# Autodesk Inventor assembly: Сборка сортировщика
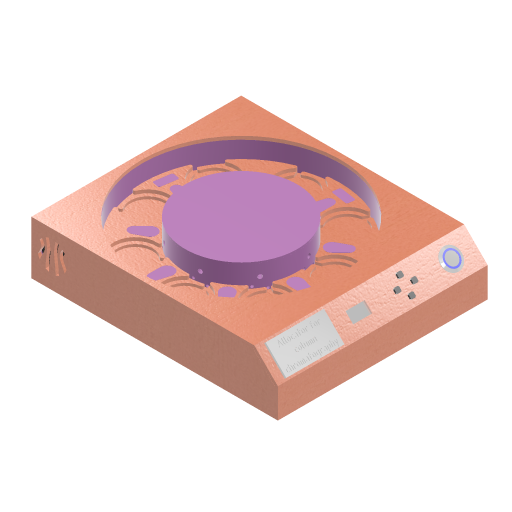
[picture p0: Inventor's stored thumbnail of the model, 512x512]
Saved by Autodesk Inventor 2024.1 (Build 281209000, 209)
## iProperties
Created: 2023-06-10
Part Number: Сборка сортировщика
Document SubType Name: Assembly
Designer: Admin
Mass: 1926.82 g
Surface Area: 9393.72 cm^2
Volume: 1926.82 cm^3
Density: 1 g/cm^3
Author: Admin
## Documents named in this file (27)
- C:\Users\aleks\OneDrive\Рабочий стол\Хроматографический сортировщик\Детали\Сборка сортировщика.iam
- C:\Users\aleks\OneDrive\Рабочий стол\Хроматографический сортировщик\Детали\Барабан в сборке.iam
- C:\Users\aleks\OneDrive\Рабочий стол\Хроматографический сортировщик\Детали\Корпус.ipt
- C:\Users\aleks\OneDrive\Рабочий стол\Хроматографический сортировщик\Детали\Покупные\Болт М3 12 мм.ipt
- C:\Users\aleks\OneDrive\Рабочий стол\Хроматографический сортировщик\Детали\Держатель динамика.ipt
- C:\Users\aleks\OneDrive\Рабочий стол\Хроматографический сортировщик\Детали\Лазерная установка.ipt
- C:\Users\aleks\OneDrive\Рабочий стол\Хроматографический сортировщик\Детали\Установка датчика холла.ipt
- C:\Users\aleks\OneDrive\Рабочий стол\Хроматографический сортировщик\Детали\Концентратор.ipt
- C:\Users\aleks\OneDrive\Рабочий стол\Хроматографический сортировщик\Детали\Покупные\Мотор.ipt
- C:\Users\aleks\OneDrive\Рабочий стол\Хроматографический сортировщик\Детали\Покупные\Плата главная.ipt
- C:\Users\aleks\OneDrive\Рабочий стол\Хроматографический сортировщик\Детали\Покупные\Болт М3 35мм.ipt
- C:\Users\aleks\OneDrive\Рабочий стол\Хроматографический сортировщик\Детали\Покупные\Болт М3 16 мм.ipt
- C:\Users\aleks\OneDrive\Рабочий стол\Хроматографический сортировщик\Детали\Покупные\Подшипник.ipt
- C:\Users\aleks\OneDrive\Рабочий стол\Хроматографический сортировщик\Детали\Покупные\Лазер.ipt
- C:\Users\aleks\OneDrive\Рабочий стол\Хроматографический сортировщик\Детали\Покупные\Лазер маленький.ipt
- C:\Users\aleks\OneDrive\Рабочий стол\Хроматографический сортировщик\Детали\Планетарная шестерня.ipt
- C:\Users\aleks\OneDrive\Рабочий стол\Хроматографический сортировщик\Детали\Шестерня малая.ipt
- C:\Users\aleks\OneDrive\Рабочий стол\Хроматографический сортировщик\Детали\Покупные\Вал.ipt
- C:\Users\aleks\OneDrive\Рабочий стол\Хроматографический сортировщик\Детали\Покупные\Болт М3 6 мм.ipt
- C:\Users\aleks\OneDrive\Рабочий стол\Хроматографический сортировщик\Детали\Покупные\Динамик.ipt
- C:\Users\aleks\OneDrive\Рабочий стол\Хроматографический сортировщик\Детали\Табличка.ipt
- C:\Users\aleks\OneDrive\Рабочий стол\Хроматографический сортировщик\Детали\Покупные\Кнопка.ipt
- C:\Users\aleks\OneDrive\Рабочий стол\Хроматографический сортировщик\Детали\Покупные\Дисплей.ipt
- C:\Users\aleks\OneDrive\Рабочий стол\Хроматографический сортировщик\Детали\Покупные\Разъём питания.ipt
- C:\Users\aleks\OneDrive\Рабочий стол\Хроматографический сортировщик\Детали\Покупные\Шайба М3.ipt
- C:\Users\aleks\OneDrive\Рабочий стол\Хроматографический сортировщик\Детали\Покупные\Кнопка маленькая.ipt
- C:\Users\aleks\OneDrive\Рабочий стол\Хроматографический сортировщик\Детали\Окно.ipt
## Components (67 placed, 26 different names)
1. Барабан в сборке:1 [sub-assembly] — Совмещение:1, Заподлицо:1, Касательность:1, Касательность:2, Касательность:3, Совмещение:117, Совмещение:118, ЗубчПер:2
2. Корпус:1 — Совмещение:1, Заподлицо:1, Совмещение:43, Совмещение:44, Совмещение:45, Совмещение:46, Совмещение:47, Совмещение:56, Совмещение:57, Совмещение:58, Совмещение:59, Совмещение:60, Совмещение:61, Совмещение:62, Совмещение:76, Совмещение:77, Совмещение:78, Совмещение:79, Совмещение:128, Заподлицо:43, Совмещение:129, Совмещение:133, Совмещение:134, Совмещение:142, Угол:35, Совмещение:147, Совмещение:148, Совмещение:183, Совмещение:184, Совмещение:224, Заподлицо:82, Совмещение:225, Совмещение:226, Совмещение:227, Совмещение:228, Совмещение:229, Совмещение:230, Совмещение:231, Совмещение:232, Совмещение:233, Совмещение:234, Совмещение:235, Совмещение:237, Совмещение:238, Совмещение:240, Совмещение:241, Совмещение:242, Совмещение:243, Совмещение:244, Совмещение:245, Совмещение:246, Совмещение:247, Совмещение:248, Совмещение:249, Совмещение:250, Совмещение:251, Совмещение:252, Касательность:4, Касательность:5, Совмещение:253
3. Болт М3 12 мм:1 — Совмещение:88, Совмещение:180
4. Болт М3 12 мм:2 — Совмещение:72, Совмещение:85
5. Болт М3 12 мм:3 — Совмещение:73, Совмещение:87
6. Болт М3 12 мм:4 — Совмещение:71, Совмещение:86
7. Болт М3 12 мм:5 — Совмещение:67, Совмещение:91
8. Болт М3 12 мм:6 — Совмещение:64, Совмещение:95, Совмещение:242
9. Болт М3 12 мм:7 — Совмещение:63, Совмещение:94, Совмещение:243
10. Болт М3 12 мм:8 — Совмещение:65, Совмещение:93, Совмещение:245
11. Болт М3 12 мм:9 — Совмещение:66, Совмещение:92, Совмещение:244
12. Болт М3 12 мм:10 — Совмещение:68, Совмещение:90, Совмещение:184
13. Болт М3 12 мм:17 — Совмещение:69, Совмещение:89, Совмещение:183
14. Держатель динамика:1 — Совмещение:59, Совмещение:65, Совмещение:66, Совмещение:92, Совмещение:93, Совмещение:126, Совмещение:127
15. Лазерная установка:1 — Совмещение:43, Совмещение:44, Совмещение:56, Совмещение:71, Совмещение:73, Совмещение:86, Совмещение:87, Совмещение:112, Совмещение:113, Совмещение:114, Совмещение:115, Совмещение:116, Заподлицо:41
16. Установка датчика холла:1 — Совмещение:58, Совмещение:68, Совмещение:69, Совмещение:89, Совмещение:90
17. Держатель динамика:2 — Совмещение:57, Совмещение:63, Совмещение:64, Совмещение:94, Совмещение:95, Совмещение:124, Совмещение:125
18. Концентратор:1 — Совмещение:47, Совмещение:61, Совмещение:67, Совмещение:91, Совмещение:111, Заподлицо:39
19. Концентратор:2 — Совмещение:46, Совмещение:60, Совмещение:88, Совмещение:109, Заподлицо:38, Совмещение:180
20. Концентратор:3 — Совмещение:45, Совмещение:62, Совмещение:72, Совмещение:85, Совмещение:110, Заподлицо:40
21. Мотор:1 — Совмещение:76, Совмещение:96, Совмещение:97, Совмещение:98, Совмещение:99, Совмещение:100, Совмещение:101, Совмещение:102, Совмещение:103, Совмещение:119, Совмещение:120
22. Плата главная:1 — Совмещение:77, Совмещение:78, Совмещение:79, Совмещение:104, Совмещение:105, Совмещение:106, Совмещение:107, Совмещение:108
23. Болт М3 35мм:1 — Совмещение:98, Совмещение:102, Касательность:4, Совмещение:253
24. Болт М3 35мм:2 — Совмещение:97, Совмещение:101, Касательность:5
25. Болт М3 35мм:3 — Совмещение:96, Совмещение:100
26. Болт М3 35мм:4 — Совмещение:99, Совмещение:103
27. Болт М3 16 мм:1 — Совмещение:107, Заподлицо:35, Заподлицо:37, Совмещение:108
28. Болт М3 16 мм:2 — Совмещение:106, Заподлицо:35
29. Болт М3 16 мм:3 — Совмещение:105, Заподлицо:36
30. Болт М3 16 мм:4 — Совмещение:104, Заподлицо:36, Заподлицо:37
31. Подшипник:1 — Совмещение:109, Заподлицо:38, Касательность:1
32. Подшипник:2 — Совмещение:111, Заподлицо:39, Касательность:2
33. Подшипник:3 — Совмещение:110, Заподлицо:40, Касательность:3
34. Лазер:1 — Совмещение:112, Заподлицо:41
35. Лазер маленький:1 — Совмещение:114, Совмещение:115
36. Лазер маленький:2 — Совмещение:113, Совмещение:116
37. Планетарная шестерня:1 — Совмещение:117, Совмещение:118, Заподлицо:42, ЗубчПер:2, ЗубчПер:3
38. Шестерня малая:1 — Заподлицо:42, Совмещение:121, Угол:34, Совмещение:122, ЗубчПер:3
39. Вал:1 — Совмещение:119, Совмещение:120, Совмещение:121, Угол:34, Совмещение:123
40. Болт М3 6 мм:1 — Совмещение:122, Совмещение:123
41. Динамик:1 — Совмещение:126, Совмещение:127
42. Динамик:2 — Совмещение:124, Совмещение:125
43. Табличка:1 — Совмещение:128, Заподлицо:43, Совмещение:129
44. Кнопка:1 — Совмещение:133, Совмещение:134
45. Дисплей:1 — Совмещение:233, Совмещение:234, Совмещение:235, Совмещение:236
46. Разъём питания:1 — Совмещение:147, Совмещение:148
47. Болт М3 12 мм:18 — Заподлицо:71, Совмещение:216, Совмещение:251
48. Болт М3 12 мм:19 — Заподлицо:67, Заподлицо:68, Совмещение:222, Совмещение:223, Совмещение:247
49. Болт М3 12 мм:20
50. Болт М3 12 мм:21 — Заподлицо:69, Заподлицо:70, Совмещение:213, Совмещение:214, Совмещение:250
51. Болт М3 12 мм:22 — Заподлицо:70, Заподлицо:71, Совмещение:215, Совмещение:252
52. Болт М3 12 мм:23 — Заподлицо:67, Совмещение:218, Совмещение:246
53. Болт М3 12 мм:24 — Заподлицо:68, Заподлицо:69, Совмещение:217, Заподлицо:76, Совмещение:248
54. Шайба М3:1 — Совмещение:222, Совмещение:223, Заподлицо:78
55. Шайба М3:2 — Совмещение:213, Совмещение:214, Заподлицо:77
56. Шайба М3:3 — Заподлицо:74, Заподлицо:75, Совмещение:221
57. Шайба М3:4 — Заподлицо:75, Совмещение:218, Заподлицо:78, Совмещение:224
58. Шайба М3:5 — Заподлицо:73, Заподлицо:74, Совмещение:217
59. Шайба М3:6 — Заподлицо:72, Заподлицо:73, Совмещение:216, Заподлицо:77
60. Шайба М3:7 — Заподлицо:72, Совмещение:215
61. Болт М3 12 мм:25 — Совмещение:221, Заподлицо:76, Совмещение:249
62. Кнопка маленькая:1 — Заподлицо:79, Заподлицо:80, Заподлицо:81, Совмещение:227, Совмещение:228
63. Кнопка маленькая:2 — Заподлицо:79, Совмещение:229, Совмещение:230
64. Кнопка маленькая:3 — Заподлицо:81, Заподлицо:82, Совмещение:225, Совмещение:226
65. Кнопка маленькая:4 — Заподлицо:80, Совмещение:231, Совмещение:232
66. Окно:1 — Совмещение:239, Совмещение:240, Совмещение:241
67. Окно:2 — Совмещение:236, Совмещение:237, Совмещение:238, Совмещение:239
## Relationships (154: Mate 119, Flush 26, Tangent 5, Angle 2, RelateRotation 2)
- Совмещение:1 [Mate]: Барабан в сборке:1 ↔ Корпус:1
- Заподлицо:1 [Flush] (-50 mm): Барабан в сборке:1 ↔ Корпус:1
- Совмещение:43 [Mate]: Корпус:1 ↔ Лазерная установка:1
- Совмещение:44 [Mate]: Корпус:1 ↔ Лазерная установка:1
- Совмещение:45 [Mate]: Корпус:1 ↔ Концентратор:3
- Совмещение:46 [Mate]: Корпус:1 ↔ Концентратор:2
- Совмещение:47 [Mate]: Корпус:1 ↔ Концентратор:1
- Совмещение:56 [Mate]: Корпус:1 ↔ Лазерная установка:1
- Совмещение:57 [Mate]: Корпус:1 ↔ Держатель динамика:2
- Совмещение:58 [Mate]: Корпус:1 ↔ Установка датчика холла:1
- Совмещение:59 [Mate]: Корпус:1 ↔ Держатель динамика:1
- Совмещение:60 [Mate]: Корпус:1 ↔ Концентратор:2
- Совмещение:61 [Mate]: Корпус:1 ↔ Концентратор:1
- Совмещение:62 [Mate]: Корпус:1 ↔ Концентратор:3
- Совмещение:63 [Mate]: Болт М3 12 мм:7 ↔ Держатель динамика:2
- Совмещение:64 [Mate]: Болт М3 12 мм:6 ↔ Держатель динамика:2
- Совмещение:65 [Mate]: Болт М3 12 мм:8 ↔ Держатель динамика:1
- Совмещение:66 [Mate]: Болт М3 12 мм:9 ↔ Держатель динамика:1
- Совмещение:67 [Mate]: Болт М3 12 мм:5 ↔ Концентратор:1
- Совмещение:68 [Mate]: Болт М3 12 мм:10 ↔ Установка датчика холла:1
- Совмещение:69 [Mate]: Болт М3 12 мм:17 ↔ Установка датчика холла:1
- Совмещение:71 [Mate]: Болт М3 12 мм:4 ↔ Лазерная установка:1
- Совмещение:72 [Mate]: Болт М3 12 мм:2 ↔ Концентратор:3
- Совмещение:73 [Mate]: Болт М3 12 мм:3 ↔ Лазерная установка:1
- Совмещение:76 [Mate]: Корпус:1 ↔ Мотор:1
- Совмещение:77 [Mate]: Корпус:1 ↔ Плата главная:1
- Совмещение:78 [Mate]: Корпус:1 ↔ Плата главная:1
- Совмещение:79 [Mate] (6 mm): Корпус:1 ↔ Плата главная:1
- Совмещение:85 [Mate]: Болт М3 12 мм:2 ↔ Концентратор:3
- Совмещение:86 [Mate]: Болт М3 12 мм:4 ↔ Лазерная установка:1
- Совмещение:87 [Mate]: Болт М3 12 мм:3 ↔ Лазерная установка:1
- Совмещение:88 [Mate]: Болт М3 12 мм:1 ↔ Концентратор:2
- Совмещение:89 [Mate]: Болт М3 12 мм:17 ↔ Установка датчика холла:1
- Совмещение:90 [Mate]: Болт М3 12 мм:10 ↔ Установка датчика холла:1
- Совмещение:91 [Mate]: Болт М3 12 мм:5 ↔ Концентратор:1
- Совмещение:92 [Mate]: Болт М3 12 мм:9 ↔ Держатель динамика:1
- Совмещение:93 [Mate]: Болт М3 12 мм:8 ↔ Держатель динамика:1
- Совмещение:94 [Mate]: Болт М3 12 мм:7 ↔ Держатель динамика:2
- Совмещение:95 [Mate]: Болт М3 12 мм:6 ↔ Держатель динамика:2
- Совмещение:96 [Mate]: Мотор:1 ↔ Болт М3 35мм:3
- Совмещение:97 [Mate]: Мотор:1 ↔ Болт М3 35мм:2
- Совмещение:98 [Mate]: Мотор:1 ↔ Болт М3 35мм:1
- Совмещение:99 [Mate]: Мотор:1 ↔ Болт М3 35мм:4
- Совмещение:100 [Mate]: Мотор:1 ↔ Болт М3 35мм:3
- Совмещение:101 [Mate]: Мотор:1 ↔ Болт М3 35мм:2
- Совмещение:102 [Mate]: Мотор:1 ↔ Болт М3 35мм:1
- Совмещение:103 [Mate]: Мотор:1 ↔ Болт М3 35мм:4
- Совмещение:104 [Mate]: Плата главная:1 ↔ Болт М3 16 мм:4
- Совмещение:105 [Mate]: Плата главная:1 ↔ Болт М3 16 мм:3
- Совмещение:106 [Mate]: Плата главная:1 ↔ Болт М3 16 мм:2
- Совмещение:107 [Mate]: Плата главная:1 ↔ Болт М3 16 мм:1
- Заподлицо:35 [Flush]: Болт М3 16 мм:1 ↔ Болт М3 16 мм:2
- Заподлицо:36 [Flush]: Болт М3 16 мм:3 ↔ Болт М3 16 мм:4
- Заподлицо:37 [Flush]: Болт М3 16 мм:1 ↔ Болт М3 16 мм:4
- Совмещение:108 [Mate]: Плата главная:1 ↔ Болт М3 16 мм:1
- Совмещение:109 [Mate]: Концентратор:2 ↔ Подшипник:1
- Совмещение:110 [Mate]: Концентратор:3 ↔ Подшипник:3
- Совмещение:111 [Mate]: Концентратор:1 ↔ Подшипник:2
- Заподлицо:38 [Flush]: Концентратор:2 ↔ Подшипник:1
- Заподлицо:39 [Flush]: Концентратор:1 ↔ Подшипник:2
- Заподлицо:40 [Flush]: Концентратор:3 ↔ Подшипник:3
- Касательность:1 [Tangent]: Барабан в сборке:1 ↔ Подшипник:1
- Касательность:2 [Tangent]: Барабан в сборке:1 ↔ Подшипник:2
- Касательность:3 [Tangent]: Барабан в сборке:1 ↔ Подшипник:3
- Совмещение:112 [Mate]: Лазерная установка:1 ↔ Лазер:1
- Совмещение:113 [Mate]: Лазерная установка:1 ↔ Лазер маленький:2
- Совмещение:114 [Mate]: Лазерная установка:1 ↔ Лазер маленький:1
- Совмещение:115 [Mate]: Лазерная установка:1 ↔ Лазер маленький:1
- Совмещение:116 [Mate]: Лазерная установка:1 ↔ Лазер маленький:2
- Заподлицо:41 [Flush]: Лазерная установка:1 ↔ Лазер:1
- Совмещение:117 [Mate]: Барабан в сборке:1 ↔ Планетарная шестерня:1
- Совмещение:118 [Mate]: Барабан в сборке:1 ↔ Планетарная шестерня:1
- Заподлицо:42 [Flush]: Планетарная шестерня:1 ↔ Шестерня малая:1
- Совмещение:119 [Mate]: Мотор:1 ↔ Вал:1
- Совмещение:120 [Mate]: Мотор:1 ↔ Вал:1
- Совмещение:121 [Mate]: Шестерня малая:1 ↔ Вал:1
- Угол:34 [Angle] (180 deg): Шестерня малая:1 ↔ Вал:1
- Совмещение:122 [Mate]: Шестерня малая:1 ↔ Болт М3 6 мм:1
- Совмещение:123 [Mate]: Вал:1 ↔ Болт М3 6 мм:1
- ЗубчПер:2 [RelateRotation] (1 ul): Барабан в сборке:1 ↔ Планетарная шестерня:1
- Совмещение:124 [Mate]: Держатель динамика:2 ↔ Динамик:2
- Совмещение:125 [Mate]: Держатель динамика:2 ↔ Динамик:2
- Совмещение:126 [Mate]: Держатель динамика:1 ↔ Динамик:1
- Совмещение:127 [Mate]: Держатель динамика:1 ↔ Динамик:1
- Совмещение:128 [Mate]: Корпус:1 ↔ Табличка:1
- Заподлицо:43 [Flush] (10 mm): Корпус:1 ↔ Табличка:1
- Совмещение:129 [Mate]: Корпус:1 ↔ Табличка:1
- Совмещение:133 [Mate]: Корпус:1 ↔ Кнопка:1
- Совмещение:134 [Mate]: Корпус:1 ↔ Кнопка:1
- Совмещение:142 [Mate]: Корпус:1
- Угол:35 [Angle] (0 deg): Корпус:1
- ЗубчПер:3 [RelateRotation] (0.375 ul): Планетарная шестерня:1 ↔ Шестерня малая:1
- Совмещение:147 [Mate]: Корпус:1 ↔ Разъём питания:1
- Совмещение:148 [Mate]: Корпус:1 ↔ Разъём питания:1
- Совмещение:180 [Mate]: Болт М3 12 мм:1 ↔ Концентратор:2
- Совмещение:183 [Mate]: Корпус:1 ↔ Болт М3 12 мм:17
- Совмещение:184 [Mate]: Корпус:1 ↔ Болт М3 12 мм:10
- Заподлицо:67 [Flush]: Болт М3 12 мм:19 ↔ Болт М3 12 мм:23
- Заподлицо:68 [Flush]: Болт М3 12 мм:19 ↔ Болт М3 12 мм:24
- Заподлицо:69 [Flush]: Болт М3 12 мм:21 ↔ Болт М3 12 мм:24
- Заподлицо:70 [Flush]: Болт М3 12 мм:21 ↔ Болт М3 12 мм:22
- Заподлицо:71 [Flush]: Болт М3 12 мм:18 ↔ Болт М3 12 мм:22
- Заподлицо:72 [Flush]: Шайба М3:6 ↔ Шайба М3:7
- Заподлицо:73 [Flush]: Шайба М3:5 ↔ Шайба М3:6
- Заподлицо:74 [Flush]: Шайба М3:3 ↔ Шайба М3:5
- Заподлицо:75 [Flush]: Шайба М3:3 ↔ Шайба М3:4
- Совмещение:213 [Mate]: Болт М3 12 мм:21 ↔ Шайба М3:2
- Совмещение:214 [Mate]: Болт М3 12 мм:21 ↔ Шайба М3:2
- Совмещение:215 [Mate]: Болт М3 12 мм:22 ↔ Шайба М3:7
- Совмещение:216 [Mate]: Болт М3 12 мм:18 ↔ Шайба М3:6
- Совмещение:217 [Mate]: Болт М3 12 мм:24 ↔ Шайба М3:5
- Совмещение:218 [Mate]: Болт М3 12 мм:23 ↔ Шайба М3:4
- Совмещение:221 [Mate]: Шайба М3:3 ↔ Болт М3 12 мм:25
- Заподлицо:76 [Flush]: Болт М3 12 мм:24 ↔ Болт М3 12 мм:25
- Заподлицо:77 [Flush]: Шайба М3:2 ↔ Шайба М3:6
- Совмещение:222 [Mate]: Болт М3 12 мм:19 ↔ Шайба М3:1
- Совмещение:223 [Mate]: Болт М3 12 мм:19 ↔ Шайба М3:1
- Заподлицо:78 [Flush]: Шайба М3:1 ↔ Шайба М3:4
- Совмещение:224 [Mate]: Корпус:1 ↔ Шайба М3:4
- Заподлицо:79 [Flush]: Кнопка маленькая:1 ↔ Кнопка маленькая:2
- Заподлицо:80 [Flush]: Кнопка маленькая:1 ↔ Кнопка маленькая:4
- Заподлицо:81 [Flush]: Кнопка маленькая:1 ↔ Кнопка маленькая:3
- Заподлицо:82 [Flush] (1 mm): Корпус:1 ↔ Кнопка маленькая:3
- Совмещение:225 [Mate]: Корпус:1 ↔ Кнопка маленькая:3
- Совмещение:226 [Mate]: Корпус:1 ↔ Кнопка маленькая:3
- Совмещение:227 [Mate]: Корпус:1 ↔ Кнопка маленькая:1
- Совмещение:228 [Mate]: Корпус:1 ↔ Кнопка маленькая:1
- Совмещение:229 [Mate]: Корпус:1 ↔ Кнопка маленькая:2
- Совмещение:230 [Mate]: Корпус:1 ↔ Кнопка маленькая:2
- Совмещение:231 [Mate]: Корпус:1 ↔ Кнопка маленькая:4
- Совмещение:232 [Mate]: Корпус:1 ↔ Кнопка маленькая:4
- Совмещение:233 [Mate]: Корпус:1 ↔ Дисплей:1
- Совмещение:234 [Mate]: Корпус:1 ↔ Дисплей:1
- Совмещение:235 [Mate]: Корпус:1 ↔ Дисплей:1
- Совмещение:236 [Mate]: Дисплей:1 ↔ Окно:2
- Совмещение:237 [Mate]: Корпус:1 ↔ Окно:2
- Совмещение:238 [Mate]: Корпус:1 ↔ Окно:2
- Совмещение:239 [Mate]: Окно:1 ↔ Окно:2
- Совмещение:240 [Mate]: Корпус:1 ↔ Окно:1
- Совмещение:241 [Mate]: Корпус:1 ↔ Окно:1
- Совмещение:242 [Mate]: Корпус:1 ↔ Болт М3 12 мм:6
- Совмещение:243 [Mate]: Корпус:1 ↔ Болт М3 12 мм:7
- Совмещение:244 [Mate]: Корпус:1 ↔ Болт М3 12 мм:9
- Совмещение:245 [Mate]: Корпус:1 ↔ Болт М3 12 мм:8
- Совмещение:246 [Mate]: Корпус:1 ↔ Болт М3 12 мм:23
- Совмещение:247 [Mate]: Корпус:1 ↔ Болт М3 12 мм:19
- Совмещение:248 [Mate]: Корпус:1 ↔ Болт М3 12 мм:24
- Совмещение:249 [Mate]: Корпус:1 ↔ Болт М3 12 мм:25
- Совмещение:250 [Mate]: Корпус:1 ↔ Болт М3 12 мм:21
- Совмещение:251 [Mate]: Корпус:1 ↔ Болт М3 12 мм:18
- Совмещение:252 [Mate]: Корпус:1 ↔ Болт М3 12 мм:22
- Касательность:4 [Tangent]: Корпус:1 ↔ Болт М3 35мм:1
- Касательность:5 [Tangent]: Корпус:1 ↔ Болт М3 35мм:2
- Совмещение:253 [Mate]: Корпус:1 ↔ Болт М3 35мм:1
